# Autodesk Inventor assembly: Z Endstop Assembly
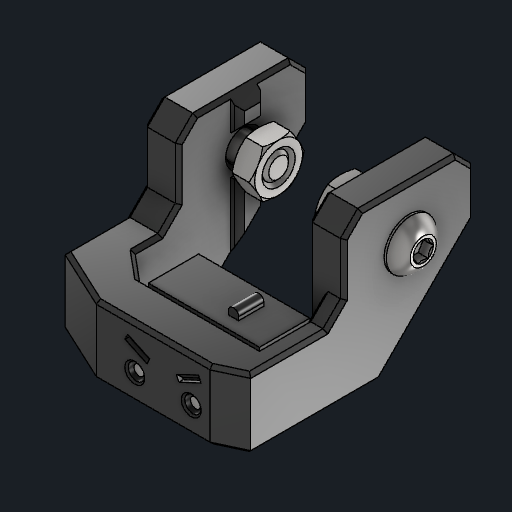
[picture p0: Inventor's stored thumbnail of the model, 512x512]
Saved by Autodesk Inventor 2026.1 (Build 301233020, 233B)
## iProperties
Created: 2025-05-09
Part Number: Z Endstop Assembly
Document SubType Name: Assembly
Designer: AdminForWorker
Title: Z Endstop Assembly
Author: AdminForWorker
## Documents named in this file (6)
- C:\Users\JoshuaEah\Documents\GitHub\Voron-0\CAD\Z Axis\Z Endstop Assembly.iam
- C:\Users\JoshuaEah\Documents\GitHub\Voron-0\CAD\Z Axis\Parts\Omron D2F Microswitch.ipt
- C:\Users\JoshuaEah\Documents\GitHub\Voron-0\CAD\Z Axis\Parts\Z Endstop Mount.ipt
- C:\Users\JoshuaEah\Documents\GitHub\Voron-0\CAD\Hardware\M2x10 Self Tapper.ipt
- C:\Users\JoshuaEah\Documents\GitHub\Voron-0\CAD\Hardware\M3x8 BHCS.ipt
- C:\Users\JoshuaEah\Documents\GitHub\Voron-0\CAD\Hardware\M3 Hexnut.ipt
## Components (8 placed, 5 different names)
1. Z Endstop Mount:1 — Insert:3, Insert:4, Insert:7, Insert:8
2. Omron D2F Microswitch:1 — Insert:1, Insert:2, Insert:3, Insert:4
3. M2x10 Self Tapping Screw:1 — Insert:2
4. M2x10 Self Tapping Screw:2 — Insert:1
5. M3x8 BHCS:1 — Insert:5, Insert:7
6. M3x8 BHCS:2 — Insert:6, Insert:8
7. M3 Hexnut:1 — Insert:5
8. M3 Hexnut:2 — Insert:6
## Relationships (8: Insert 8)
- Insert:1: Omron D2F Microswitch:1 ↔ M2x10 Self Tapping Screw:2
- Insert:2: Omron D2F Microswitch:1 ↔ M2x10 Self Tapping Screw:1
- Insert:3: Z Endstop Mount:1 ↔ Omron D2F Microswitch:1
- Insert:4: Z Endstop Mount:1 ↔ Omron D2F Microswitch:1
- Insert:5: M3x8 BHCS:1 ↔ M3 Hexnut:1
- Insert:6: M3x8 BHCS:2 ↔ M3 Hexnut:2
- Insert:7: Z Endstop Mount:1 ↔ M3x8 BHCS:1
- Insert:8: Z Endstop Mount:1 ↔ M3x8 BHCS:2
